# Autodesk Inventor assembly: Pen Holder Assembly
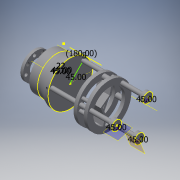
[picture p0: Inventor's stored thumbnail of the model, 180x180]
Saved by Autodesk Inventor 2019 (Build 230136000, 136)
## iProperties
Created: 2019-06-10
Part Number: Pen Holder Assembly
Document SubType Name: Assembly
Designer: Matthew XPS
Author: Matthew XPS
## Documents named in this file (8)
- G:\My Drive\Documents\Human Robot Interaction Lab\Projects\2019-06 Adept Viper Robot Arm\Pen  Holder\Pen Holder Assembly.iam
- G:\My Drive\Documents\Human Robot Interaction Lab\Projects\2019-06 Adept Viper Robot Arm\Pen  Holder\Clamp Plate.ipt
- G:\My Drive\Documents\Human Robot Interaction Lab\Projects\2019-06 Adept Viper Robot Arm\Pen  Holder\New Interface.ipt
- G:\My Drive\Documents\Human Robot Interaction Lab\Projects\2019-06 Adept Viper Robot Arm\Pen  Holder\Pen Holder Interface.ipt
- G:\My Drive\Documents\Human Robot Interaction Lab\Projects\2019-06 Adept Viper Robot Arm\Pen  Holder\Pen Main Piece.ipt
- G:\My Drive\Documents\Human Robot Interaction Lab\Projects\2019-06 Adept Viper Robot Arm\Pen  Holder\Robot Flange.ipt
- G:\My Drive\Documents\Human Robot Interaction Lab\Projects\2019-06 Adept Viper Robot Arm\Pen  Holder\6mm rod.ipt
- G:\My Drive\Documents\Human Robot Interaction Lab\Projects\2019-06 Adept Viper Robot Arm\Pen  Holder\6mm rod topper.ipt
## Components (11 placed, 7 different names)
1. Clamp Plate:1 — Rotational:1
2. New Interface:1 — Rigid:2, Rotational:2, Rotational:3, Rigid:3
3. Pen Holder Interface:1 — Rigid:3, Mate:4
4. Pen Main Piece:1 — Rotational:1, Mate:1, Mate:2, Mate:3
5. Robot Flange:1 — Mate:4
6. 6mm rod:1 — Rigid:2, Mate:1, Rigid:4
7. 6mm rod:2 — Rotational:2, Rigid:5, Mate:3
8. 6mm rod:3 — Rotational:3, Mate:2, Rigid:6
9. 6mm rod topper:1 — Rigid:4
10. 6mm rod topper:2 — Rigid:5
11. 6mm rod topper:3 — Rigid:6
## Relationships (12: WeldJoint 5, Mate 4, RevoluteJoint 3)
- Rotational:1 [RevoluteJoint] (-0.5 mm): Clamp Plate:1 ↔ Pen Main Piece:1
- Rigid:2 [WeldJoint]: New Interface:1 ↔ 6mm rod:1
- Rotational:2 [RevoluteJoint]: New Interface:1 ↔ 6mm rod:2
- Rotational:3 [RevoluteJoint]: New Interface:1 ↔ 6mm rod:3
- Mate:1: Pen Main Piece:1 ↔ 6mm rod:1
- Mate:2: Pen Main Piece:1 ↔ 6mm rod:3
- Rigid:3 [WeldJoint]: New Interface:1 ↔ Pen Holder Interface:1
- Rigid:4 [WeldJoint]: 6mm rod:1 ↔ 6mm rod topper:1
- Rigid:5 [WeldJoint]: 6mm rod:2 ↔ 6mm rod topper:2
- Rigid:6 [WeldJoint]: 6mm rod:3 ↔ 6mm rod topper:3
- Mate:3: Pen Main Piece:1 ↔ 6mm rod:2
- Mate:4: Pen Holder Interface:1 ↔ Robot Flange:1
